# Autodesk Inventor assembly: AxisX
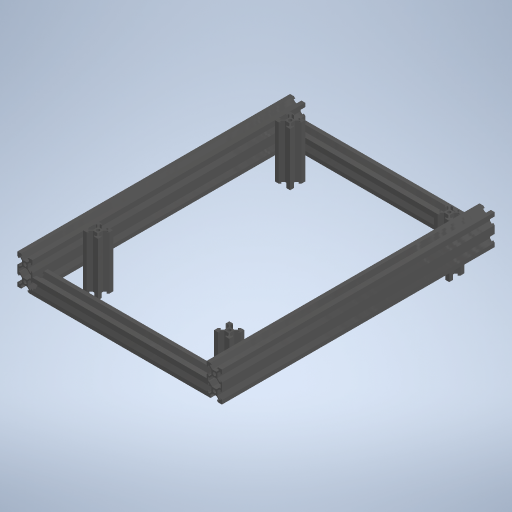
[picture p0: Inventor's stored thumbnail of the model, 512x512]
Saved by Autodesk Inventor 2024.2 (Build 282272000, 272)
## iProperties
Created: 2024-08-26
Part Number: AxisX
Document SubType Name: Assembly
Designer: Admin
Author: Admin
## Documents named in this file (4)
- C:\Users\Admin\Documents\GitHub\RobotCartesiano\DiseñoBrazo\Assemblies\AxisX.iam
- C:\Users\Admin\Documents\GitHub\RobotCartesiano\DiseñoBrazo\AluminumProfiles\AxisX\AP-X1.ipt
- C:\Users\Admin\Documents\GitHub\RobotCartesiano\DiseñoBrazo\AluminumProfiles\AxisX\AP-X2.ipt
- C:\Users\Admin\Documents\GitHub\RobotCartesiano\DiseñoBrazo\AluminumProfiles\AxisX\AP-Support.ipt
## Components (8 placed, 3 different names)
1. AP-X1:1 — Mate:1, Flush:1, Flush:2, Mate:3, Flush:5, Flush:8, Mate:7
2. AP-X1:2 — Mate:2, Flush:3, Flush:4, Mate:4, Flush:6, Mate:6, Flush:7, Flush:9
3. AP-X2:1 — Mate:3, Mate:4, Flush:5, Flush:6, Mate:5, Mate:8
4. AP-X2:2 — Mate:1, Flush:1, Flush:2, Mate:2, Flush:3, Flush:4
5. AP-Support:1 — Mate:5, Mate:6, Flush:7
6. AP-Support:2 — Flush:9
7. AP-Support:3
8. AP-Support:4 — Flush:8, Mate:7, Mate:8
## Relationships (17: Flush 9, Mate 8)
- Mate:1: AP-X1:1 ↔ AP-X2:2
- Flush:1: AP-X1:1 ↔ AP-X2:2
- Flush:2: AP-X1:1 ↔ AP-X2:2
- Mate:2: AP-X1:2 ↔ AP-X2:2
- Flush:3: AP-X1:2 ↔ AP-X2:2
- Flush:4: AP-X1:2 ↔ AP-X2:2
- Mate:3: AP-X1:1 ↔ AP-X2:1
- Mate:4: AP-X1:2 ↔ AP-X2:1
- Flush:5: AP-X1:1 ↔ AP-X2:1
- Flush:6: AP-X1:2 ↔ AP-X2:1
- Mate:5: AP-X2:1 ↔ AP-Support:1
- Mate:6: AP-X1:2 ↔ AP-Support:1
- Flush:7: AP-X1:2 ↔ AP-Support:1
- Flush:8: AP-X1:1 ↔ AP-Support:4
- Mate:7: AP-X1:1 ↔ AP-Support:4
- Mate:8: AP-X2:1 ↔ AP-Support:4
- Flush:9: AP-X1:2 ↔ AP-Support:2
